# Autodesk Inventor assembly: Camera Assembly
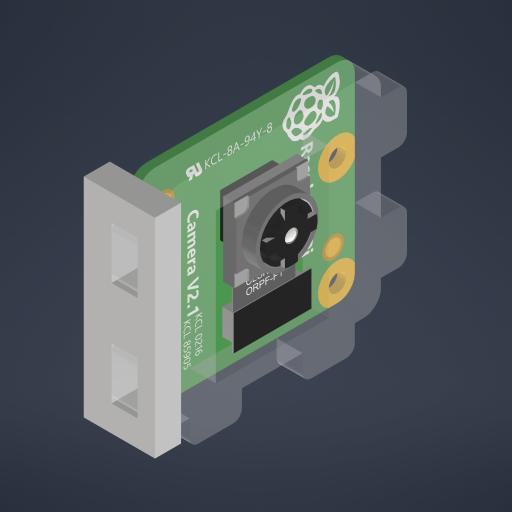
[picture p0: Inventor's stored thumbnail of the model, 512x512]
Saved by Autodesk Inventor 2023 (Build 270158000, 158)
## iProperties
Created: 2023-03-14
Part Number: Camera Assembly
Document SubType Name: Assembly
Designer: Matt
Author: Matt
## Documents named in this file (4)
- C:\Users\Matt\Documents\ROBOTS101_CAD\1. CAD MODELS\Pi Cam\Camera Holder\Camera Assembly.iam
- C:\Users\Matt\Documents\ROBOTS101_CAD\1. CAD MODELS\Pi Cam\Cam V2.1 v1.ipt
- C:\Users\Matt\Documents\ROBOTS101_CAD\1. CAD MODELS\Pi Cam\Camera Holder\FacePlate.ipt
- C:\Users\Matt\Documents\ROBOTS101_CAD\1. CAD MODELS\Pi Cam\Camera Holder\SideClip.ipt
## Components (3 placed, 3 different names)
1. Cam V2.1 v1:1 — Mate:1, Flush:1, Flush:2
2. FacePlate:1 — Mate:1, Flush:1, Flush:2, Mate:2, Mate:3, Mate:4
3. SideClip:1 — Mate:2, Mate:3, Mate:4
## Relationships (6: Mate 4, Flush 2)
- Mate:1: Cam V2.1 v1:1 ↔ FacePlate:1
- Flush:1: Cam V2.1 v1:1 ↔ FacePlate:1
- Flush:2: Cam V2.1 v1:1 ↔ FacePlate:1
- Mate:2: FacePlate:1 ↔ SideClip:1
- Mate:3: FacePlate:1 ↔ SideClip:1
- Mate:4: FacePlate:1 ↔ SideClip:1
